# Autodesk Inventor assembly: ASY PNS waste water bin 00
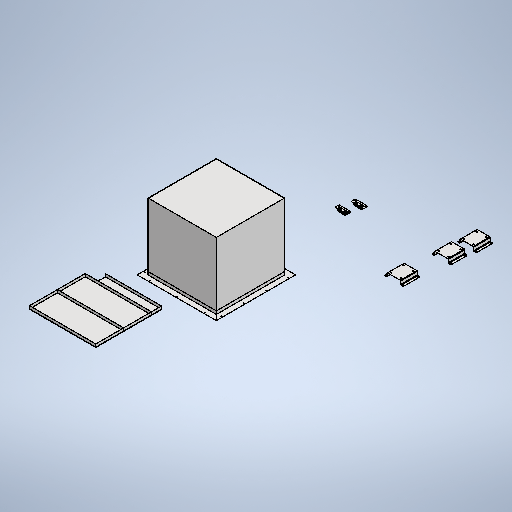
[picture p0: Inventor's stored thumbnail of the model, 512x512]
Saved by Autodesk Inventor 2025.3 (Build 293356030, 356C)
## iProperties
Created: 2025-09-03
Part Number: ASY PNS waste water bin 00
Document SubType Name: Assembly
Designer: admin
Author: admin
## Documents named in this file (13)
- C:\Users\admin\Yandex.Disk\home pc\Inventor\PNS2-Panaevsk\ASY PNS waste water bin 00.iam
- C:\Users\admin\Yandex.Disk\home pc\Inventor\PNS2-Panaevsk\PNS waste water bin 01.ipt
- C:\Users\admin\Yandex.Disk\home pc\Inventor\PNS2-Panaevsk\motor pillar 1.ipt
- C:\Users\admin\Yandex.Disk\home pc\Inventor\PNS2-Panaevsk\motor pillar 2.ipt
- C:\Users\admin\Yandex.Disk\home pc\Inventor\PNS2-Panaevsk\motor pillar 4.ipt
- C:\Users\admin\Yandex.Disk\home pc\Inventor\PNS2-Panaevsk\PNS waste water bin 02.ipt
- C:\Users\admin\Yandex.Disk\home pc\Inventor\PNS2-Panaevsk\PNS waste water bin 03.ipt
- C:\Users\admin\Yandex.Disk\home pc\Inventor\PNS2-Panaevsk\PNS waste water bin 04.ipt
- C:\Users\admin\Yandex.Disk\home pc\Inventor\PNS2-Panaevsk\PNS waste water bin 06.ipt
- C:\Users\admin\Yandex.Disk\home pc\Inventor\PNS2-Panaevsk\PNS waste water bin 07.ipt
- C:\Users\admin\Yandex.Disk\home pc\Inventor\PNS2-Panaevsk\PNS waste water bin 08.ipt
- C:\Users\admin\Yandex.Disk\home pc\Inventor\PNS2-Panaevsk\PNS waste water bin 09.ipt
- C:\Users\admin\Yandex.Disk\home pc\Inventor\PNS2-Panaevsk\PNS- motor 030 reductor pillar.ipt
## Components (35 placed, 12 different names)
1. PNS waste water bin 01:1 — Rigid:15, Rigid:17, Rigid:18
2. motor pillar 1:1 — Rigid:1
3. motor pillar 2:1 — Rigid:1, Rigid:2
4. motor pillar 2:2 — Rigid:2, Rigid:3
5. motor pillar 2:3 — Rigid:3, Rigid:4
6. motor pillar 2:4 — Rigid:4, Rigid:6
7. motor pillar 2:5 — Rigid:6
8. motor pillar 2:6 — Rigid:7
9. motor pillar 4:1 — Rigid:7
10. motor pillar 1:2
11. motor pillar 2:7
12. motor pillar 2:8
13. motor pillar 2:9
14. motor pillar 2:10
15. motor pillar 2:11
16. motor pillar 2:12
17. motor pillar 4:2
18. PNS waste water bin 01:2 — Rigid:15, Rigid:16, Rigid:19, Flush:1
19. PNS waste water bin 02:1 — Rigid:16, Rigid:20, Mate:1
20. PNS waste water bin 02:2 — Rigid:17
21. PNS waste water bin 03:1 — Rigid:18
22. PNS waste water bin 03:2 — Rigid:19, Mate:2
23. PNS waste water bin 04:1 — Rigid:20
24. PNS waste water bin 06:1 — Rigid:22
25. PNS waste water bin 06:2 — Rigid:22, Mate:1, Mate:2, Flush:1
26. PNS waste water bin 07:1 — Rigid:23, Rigid:24, Rigid:25
27. PNS waste water bin 08:1 — Rigid:23
28. PNS waste water bin 09:1 — Rigid:24
29. PNS waste water bin 09:2 — Rigid:25, Rigid:26, Rigid:27, Rigid:28
30. PNS waste water bin 08:2 — Rigid:26
31. PNS waste water bin 08:3 — Rigid:27
32. PNS waste water bin 08:4 — Rigid:28
33. Part1:1
34. Part1:2
35. Part1:3
## Relationships (30: WeldJoint 27, Mate 2, Flush 1)
- Rigid:1 [WeldJoint]: motor pillar 1:1 ↔ motor pillar 2:1
- Rigid:2 [WeldJoint]: motor pillar 2:1 ↔ motor pillar 2:2
- Rigid:3 [WeldJoint]: motor pillar 2:2 ↔ motor pillar 2:3
- Rigid:4 [WeldJoint]: motor pillar 2:3 ↔ motor pillar 2:4
- [WeldJoint]: motor pillar 2:5 ↔ motor pillar 2:6
- Rigid:6 [WeldJoint]: motor pillar 2:4 ↔ motor pillar 2:5
- Rigid:7 [WeldJoint]: motor pillar 2:6 ↔ motor pillar 4:1
- [WeldJoint]: motor pillar 1:2 ↔ motor pillar 2:7
- [WeldJoint]: motor pillar 2:7 ↔ motor pillar 2:8
- [WeldJoint]: motor pillar 2:8 ↔ motor pillar 2:9
- [WeldJoint]: motor pillar 2:9 ↔ motor pillar 2:10
- [WeldJoint]: motor pillar 2:11 ↔ motor pillar 2:12
- [WeldJoint]: motor pillar 2:10 ↔ motor pillar 2:11
- [WeldJoint]: motor pillar 2:12 ↔ motor pillar 4:2
- Rigid:15 [WeldJoint]: PNS waste water bin 01:1 ↔ PNS waste water bin 01:2
- Rigid:16 [WeldJoint]: PNS waste water bin 01:2 ↔ PNS waste water bin 02:1
- Rigid:17 [WeldJoint]: PNS waste water bin 01:1 ↔ PNS waste water bin 02:2
- Rigid:18 [WeldJoint]: PNS waste water bin 01:1 ↔ PNS waste water bin 03:1
- Rigid:19 [WeldJoint]: PNS waste water bin 01:2 ↔ PNS waste water bin 03:2
- Rigid:20 [WeldJoint]: PNS waste water bin 02:1 ↔ PNS waste water bin 04:1
- Rigid:22 [WeldJoint]: PNS waste water bin 06:1 ↔ PNS waste water bin 06:2
- Mate:1: PNS waste water bin 02:1 ↔ PNS waste water bin 06:2
- Mate:2: PNS waste water bin 03:2 ↔ PNS waste water bin 06:2
- Flush:1 (20 mm): PNS waste water bin 01:2 ↔ PNS waste water bin 06:2
- Rigid:23 [WeldJoint]: PNS waste water bin 07:1 ↔ PNS waste water bin 08:1
- Rigid:24 [WeldJoint]: PNS waste water bin 07:1 ↔ PNS waste water bin 09:1
- Rigid:25 [WeldJoint]: PNS waste water bin 07:1 ↔ PNS waste water bin 09:2
- Rigid:26 [WeldJoint]: PNS waste water bin 09:2 ↔ PNS waste water bin 08:2
- Rigid:27 [WeldJoint]: PNS waste water bin 09:2 ↔ PNS waste water bin 08:3
- Rigid:28 [WeldJoint]: PNS waste water bin 09:2 ↔ PNS waste water bin 08:4
## Named parameters: d4_d1 = 0 mm, d7_d0 = 0 mm, d8_d1 = 0 mm, d9_d2 = 0 mm, d10_d3 = 0 mm, d11_d4_d1 = 0 mm, d12_d5 = 0 mm, d13_d6 = 0 mm
